# Autodesk Inventor assembly: MecanumAssembly
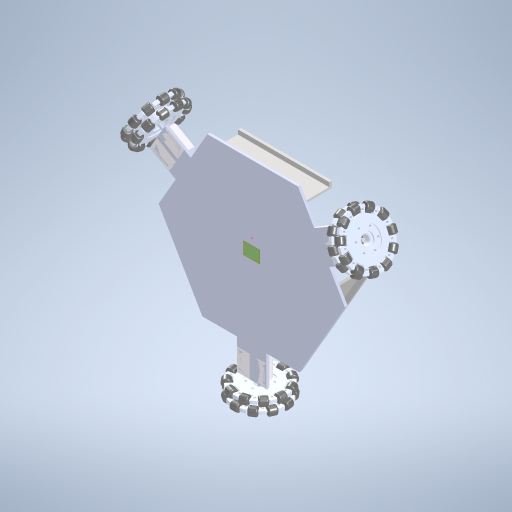
[picture p0: Inventor's stored thumbnail of the model, 512x512]
Saved by Autodesk Inventor 2024 (Build 280153000, 153)
## iProperties
Created: 2023-11-19
Part Number: MecanumAssembly
Document SubType Name: Assembly
Designer: pratikhya
Sending System: SolidWorks 2021
Last Author: mrl-iitk
Last Saved: 2023-12-06
Definition: UNKNOWN
Source: NOT_KNOWN
Part Number: Assem1
Nomenclature: Assem1
Author: pratikhya
Revision Number: ANY
## Documents named in this file (5)
- C:\Users\prati\OneDrive - IIT Kanpur\Desktop\Robot\MecanumAssembly.iam
- C:\Users\prati\Downloads\aditya\aditya\RobotAssembly\WheelStructure.ipt
- C:\Users\prati\Downloads\aditya\aditya\RobotAssembly\Assem18^MecanumAssembly.iam
- C:\Users\prati\Downloads\aditya\aditya\RobotAssembly\Assem1.iam
- C:\Users\prati\OneDrive - IIT Kanpur\Desktop\Robot\Flange.ipt
## Components (10 placed, 4 different names)
1. WheelStructure:1 — Mate:5, Flush:3, Mate:6, Flush:4, Mate:7, Flush:5
2. Assem18^MecanumAssembly:1 [sub-assembly]
3. Assem18^MecanumAssembly:2 [sub-assembly]
4. Assem18^MecanumAssembly:3 [sub-assembly]
5. Assem1:2 [sub-assembly]
6. Assem1:3 [sub-assembly]
7. Assem1:4 [sub-assembly]
8. Flange:1 — Mate:5, Flush:3
9. Flange:2 — Mate:6, Flush:4
10. Flange:3 — Mate:7, Flush:5
## Relationships (6: Mate 3, Flush 3)
- Mate:5: WheelStructure:1 ↔ Flange:1
- Flush:3 (20 mm): WheelStructure:1 ↔ Flange:1
- Mate:6: WheelStructure:1 ↔ Flange:2
- Flush:4 (20 mm): WheelStructure:1 ↔ Flange:2
- Mate:7: WheelStructure:1 ↔ Flange:3
- Flush:5 (20 mm): WheelStructure:1 ↔ Flange:3
